# Autodesk Inventor assembly: Mon30_P2_assembly
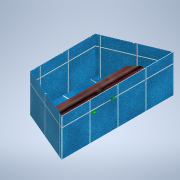
[picture p0: Inventor's stored thumbnail of the model, 180x180]
Saved by Autodesk Inventor 2021 (Build 250183000, 183)
## iProperties
Created: 2020-11-30
Part Number: Mon30_P2_assembly
Document SubType Name: Assembly
Designer: gurle
Author: gurle
## Documents named in this file (4)
- C:\Users\gurle\Downloads\Mon30_P2_assembly.iam
- C:\Users\gurle\Downloads\Scalpel Handle1.ipt
- C:\Users\gurle\Downloads\footprint.ipt
- C:\Users\gurle\Downloads\MON30_P2_Container.ipt
## Components (3 placed, 3 different names)
1. Scalpel Handle1:1 — Mate:3, Mate:4
2. footprint:1 — Mate:1, Mate:2
3. MON30_P2_Container:1 — Mate:1, Mate:2, Mate:3, Mate:4
## Relationships (4: Mate 4)
- Mate:1: footprint:1 ↔ MON30_P2_Container:1
- Mate:2: footprint:1 ↔ MON30_P2_Container:1
- Mate:3: Scalpel Handle1:1 ↔ MON30_P2_Container:1
- Mate:4: Scalpel Handle1:1 ↔ MON30_P2_Container:1
